# Autodesk Inventor assembly: base
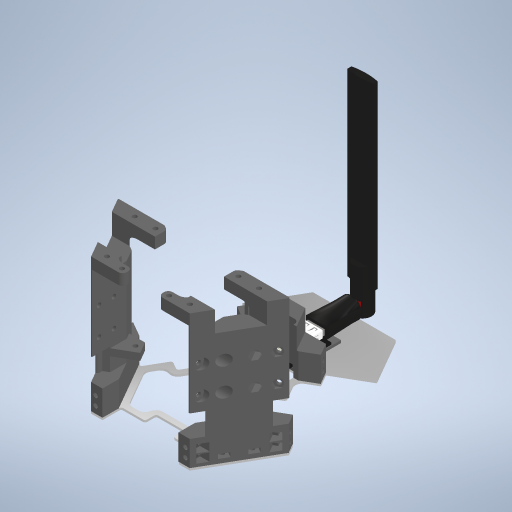
[picture p0: Inventor's stored thumbnail of the model, 512x512]
Saved by Autodesk Inventor 2024.1 (Build 281209000, 209)
## iProperties
Created: 2025-02-03
Part Number: base
Document SubType Name: Assembly
Designer: hibik
Author: hibik
## Documents named in this file (7)
- C:\Users\hibik\Documents\Robomech\RESCUE\ORCA\hard\flame_base\base.iam
- C:\Users\hibik\Documents\Robomech\RESCUE\ORCA\hard\flame_base\base_plate.ipt
- C:\Users\hibik\Documents\Robomech\RESCUE\ORCA\hard\flame_base\base_plate_towheel.ipt
- C:\Users\hibik\Documents\Robomech\RESCUE\ORCA\hard\flame_base\base_plate_towheel_front_right.ipt
- C:\Users\hibik\Documents\Robomech\RESCUE\ORCA\hard\std_parts\Buffalo_Wl-U2-433DHP.ipt
- C:\Users\hibik\Documents\Robomech\RESCUE\ORCA\hard\board\CORE_model\external_io_usbA.iam
- C:\Users\hibik\Documents\Robomech\RESCUE\ORCA\hard\flame_base\base_plate_towheel_front_right_MIR.ipt
## Components (6 placed, 6 different names)
1. base_plate:1 — 挿入:1, 挿入:2, フラッシュ:9, フラッシュ:10, メイト:1
2. base_plate_towheel:3 — フラッシュ:9, フラッシュ:10, メイト:1, 挿入:5, 角度:1
3. base_plate_towheel_front_right:1 — 挿入:1, 挿入:2
4. Buffalo_Wl-U2-433DHP:1 — メイト:2, メイト:3, フラッシュ:11
5. external_io_usbA:1 [sub-assembly] — 挿入:5, 角度:1, メイト:2, メイト:3
6. base_plate_towheel_front_right_MIR:1
## Relationships (10: Insert 3, Flush 3, Mate 3, Angle 1)
- 挿入:1 [Insert]: base_plate:1 ↔ base_plate_towheel_front_right:1
- 挿入:2 [Insert]: base_plate:1 ↔ base_plate_towheel_front_right:1
- フラッシュ:9 [Flush]: base_plate:1 ↔ base_plate_towheel:3
- フラッシュ:10 [Flush]: base_plate:1 ↔ base_plate_towheel:3
- メイト:1 [Mate]: base_plate:1 ↔ base_plate_towheel:3
- 挿入:5 [Insert] (0.5 mm): base_plate_towheel:3 ↔ external_io_usbA:1
- 角度:1 [Angle] (0 deg): base_plate_towheel:3 ↔ external_io_usbA:1
- メイト:2 [Mate] (2 mm): Buffalo_Wl-U2-433DHP:1 ↔ external_io_usbA:1
- メイト:3 [Mate] (0.5 mm): Buffalo_Wl-U2-433DHP:1 ↔ external_io_usbA:1
- フラッシュ:11 [Flush]: Buffalo_Wl-U2-433DHP:1
